# Autodesk Inventor assembly: 足全体
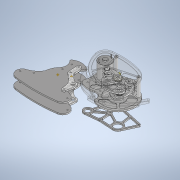
[picture p0: Inventor's stored thumbnail of the model, 180x180]
Saved by Autodesk Inventor 2022.2 (Build 262287010, 287A)
## iProperties
Created: 2022-01-30
Part Number: 足全体
Document SubType Name: Assembly
Designer: acps
Author: acps
## Documents named in this file (4)
- C:\Users\acps\Documents\srdc\srdc_ksh\脚\足全体.iam
- C:\Users\acps\Documents\srdc\srdc_ksh\脚\中間ユニット外.ipt
- C:\Users\acps\Documents\srdc\srdc_ksh\脚\アーノン.ipt
- C:\Users\acps\Documents\srdc\srdc_ksh\脚\足ユニット.iam
## Components (5 placed, 3 different names)
1. 中間ユニット外:1 — Mate:1, Mate:2, Mate:4, Mate:5, Mate:6, Mate:7
2. アーノン:1 — Mate:1, Mate:2, Mate:3
3. 足ユニット:1 [sub-assembly] — Mate:3
4. 中間ユニット外:2 — Mate:5, Mate:6
5. アーノン:2 — Mate:4, Mate:7
## Relationships (7: Mate 7)
- Mate:1: 中間ユニット外:1 ↔ アーノン:1
- Mate:2: 中間ユニット外:1 ↔ アーノン:1
- Mate:3: アーノン:1 ↔ 足ユニット:1
- Mate:4: 中間ユニット外:1 ↔ アーノン:2
- Mate:5: 中間ユニット外:1 ↔ 中間ユニット外:2
- Mate:6: 中間ユニット外:1 ↔ 中間ユニット外:2
- Mate:7: 中間ユニット外:1 ↔ アーノン:2
